# Autodesk Inventor assembly: leftInsertbearing_MIR
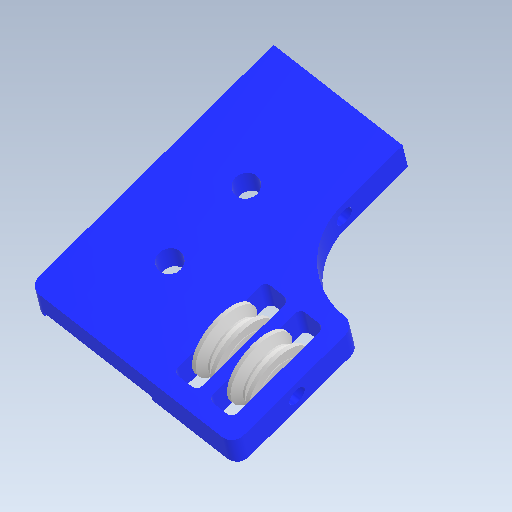
[picture p0: Inventor's stored thumbnail of the model, 512x512]
Saved by Autodesk Inventor 2020 (Build 240168000, 168)
## iProperties
Created: 2019-12-19
Part Number: leftInsertbearing_MIR
Document SubType Name: Assembly
Designer: xj82b
Author: xj82b
## Documents named in this file (3)
- C:\Users\xj82b\Documents\Inventor\5199\leftInsertbearing_MIR.iam
- C:\Users\xj82b\Documents\Inventor\5199\3x12x4mm-bearing_MIR.ipt
- C:\Users\xj82b\Documents\Inventor\5199\leftshortNEW_MIR.ipt
## Components (3 placed, 2 different names)
1. 3x12x4mm-bearing_MIR:1 — Mate:2, Mate:1
2. 3x12x4mm-bearing_MIR:2 — Mate:4, Mate:3
3. leftshortNEW_MIR:1 — Mate:4, Mate:3, Mate:2, Mate:1
## Relationships (4: Mate 4)
- Mate:4: 3x12x4mm-bearing_MIR:2 ↔ leftshortNEW_MIR:1
- Mate:3: 3x12x4mm-bearing_MIR:2 ↔ leftshortNEW_MIR:1
- Mate:2: 3x12x4mm-bearing_MIR:1 ↔ leftshortNEW_MIR:1
- Mate:1: 3x12x4mm-bearing_MIR:1 ↔ leftshortNEW_MIR:1
